# Autodesk Inventor assembly: Armor_Front
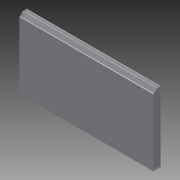
[picture p0: Inventor's stored thumbnail of the model, 180x180]
Saved by Autodesk Inventor 2013 (Build 170138000, 138)
## iProperties
Created: 2015-07-02
Part Number: Armor_Front
Document SubType Name: Assembly
Designer: Kyle
Mass: 55.2096 g
Surface Area: 636.937 cm^2
Volume: 36.6341 cm^3
Density: 1.50706 g/cm^3
Author: Kyle
## Documents named in this file (5)
- C:\Users\Kyle\Documents\Project documentation\Combat Robot\CAD\V1.0\Armor_Front.iam
- C:\Users\Kyle\Documents\Project documentation\Combat Robot\CAD\V1.0\Plate_Front_Poly.ipt
- C:\Users\Kyle\Documents\Project documentation\Combat Robot\CAD\V1.0\Plate_Front_Alu26.ipt
- C:\Users\Kyle\Documents\Project documentation\Combat Robot\CAD\V1.0\Plate_FrontChamfer_Poly.ipt
- C:\Users\Kyle\Documents\Project documentation\Combat Robot\CAD\V1.0\Plate_FrontShort_Alu26.ipt
## Components (5 placed, 4 different names)
1. Plate_Front_Poly:2 — Mate:3, Mate:4, Flush:3, Flush:4, Flush:7, Flush:8
2. Plate_Front_Alu26:2 — Mate:3, Flush:3, Flush:7, Mate:5, Flush:9, Flush:10
3. Plate_Front_Alu26:3 — Mate:4, Flush:4, Flush:8
4. Plate_FrontChamfer_Poly:1 — Mate:5, Flush:9, Flush:10, Mate:6, Flush:11, Flush:12
5. Plate_FrontShort_Alu26:1 — Mate:6, Flush:11, Flush:12
## Relationships (12: Flush 8, Mate 4)
- Mate:3: Plate_Front_Poly:2 ↔ Plate_Front_Alu26:2
- Mate:4: Plate_Front_Poly:2 ↔ Plate_Front_Alu26:3
- Flush:3: Plate_Front_Poly:2 ↔ Plate_Front_Alu26:2
- Flush:4: Plate_Front_Poly:2 ↔ Plate_Front_Alu26:3
- Flush:7: Plate_Front_Poly:2 ↔ Plate_Front_Alu26:2
- Flush:8: Plate_Front_Poly:2 ↔ Plate_Front_Alu26:3
- Mate:5: Plate_Front_Alu26:2 ↔ Plate_FrontChamfer_Poly:1
- Flush:9: Plate_Front_Alu26:2 ↔ Plate_FrontChamfer_Poly:1
- Flush:10: Plate_Front_Alu26:2 ↔ Plate_FrontChamfer_Poly:1
- Mate:6: Plate_FrontChamfer_Poly:1 ↔ Plate_FrontShort_Alu26:1
- Flush:11: Plate_FrontChamfer_Poly:1 ↔ Plate_FrontShort_Alu26:1
- Flush:12: Plate_FrontChamfer_Poly:1 ↔ Plate_FrontShort_Alu26:1
